# Autodesk Inventor assembly: esp32-devkitc-v4
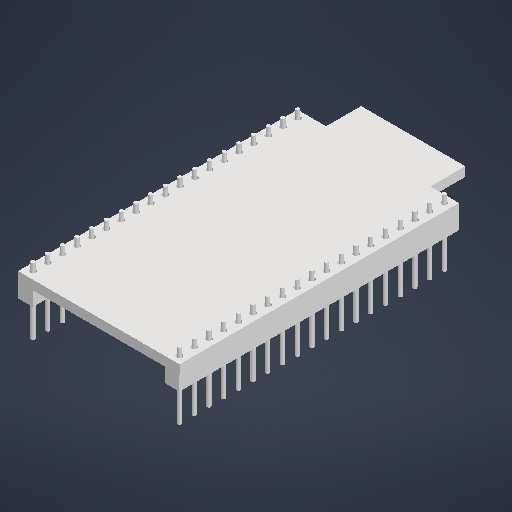
[picture p0: Inventor's stored thumbnail of the model, 512x512]
Saved by Autodesk Inventor 2025.2 (Build 292293000, 293)
## iProperties
Created: 2025-11-15
Part Number: esp32-devkitc-v4
Document SubType Name: Assembly
Designer: sam
Author: sam
## Documents named in this file (3)
- G:\projects\primary\auto-water-distribution-system\model\asm\module-command\electronic-components\esp32-devkitc-v4.iam
- G:\projects\primary\auto-water-distribution-system\model\asm\general\pin-header-male.ipt
- G:\projects\primary\auto-water-distribution-system\model\asm\module-command\electronic-components\esp32-devkitc-v4.ipt
## Components (39 placed, 2 different names)
1. esp32-devkitc-v4:1 — Mate:1, Mate:2, Mate:3, Mate:4
2. pin-header-male:1 — Mate:1, Mate:2
3. pin-header-male:2
4. pin-header-male:3
5. pin-header-male:4
6. pin-header-male:5
7. pin-header-male:6
8. pin-header-male:7
9. pin-header-male:8
10. pin-header-male:9
11. pin-header-male:10
12. pin-header-male:11
13. pin-header-male:12
14. pin-header-male:13
15. pin-header-male:14
16. pin-header-male:15
17. pin-header-male:16
18. pin-header-male:17
19. pin-header-male:18
20. pin-header-male:19
21. pin-header-male:20 — Mate:3, Mate:4
22. pin-header-male:21
23. pin-header-male:22
24. pin-header-male:23
25. pin-header-male:24
26. pin-header-male:25
27. pin-header-male:26
28. pin-header-male:27
29. pin-header-male:28
30. pin-header-male:29
31. pin-header-male:30
32. pin-header-male:31
33. pin-header-male:32
34. pin-header-male:33
35. pin-header-male:34
36. pin-header-male:35
37. pin-header-male:36
38. pin-header-male:37
39. pin-header-male:38
## Component patterns: (19 elements, first: pin-header-male:1), (19 elements, first: pin-header-male:20)
## Relationships (4: Mate 4)
- Mate:1: esp32-devkitc-v4:1 ↔ pin-header-male:1
- Mate:2: esp32-devkitc-v4:1 ↔ pin-header-male:1
- Mate:3: esp32-devkitc-v4:1 ↔ pin-header-male:20
- Mate:4: esp32-devkitc-v4:1 ↔ pin-header-male:20
